# Autodesk Inventor assembly: NEMA 17 with T5 Pulley
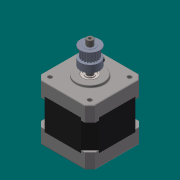
[picture p0: Inventor's stored thumbnail of the model, 180x180]
Saved by Autodesk Inventor 2016 (Build 200138000, 138)
## iProperties
Created: 2015-02-28
Part Number: NEMA 17 with T5 Pulley
Document SubType Name: Assembly
Designer: Sawaiz Syed
Title: NEMA 17 with T5 Pulley.STP
Description: STEP AP214
Creation Date: 2013-02-23
Sending System: SolidWorks 2012
Preprocessor: SwSTEP 2.0
Author: Sawaiz Syed
## Documents named in this file (8)
- C:\Users\Sawaiz\Documents\data\projects\cncBlackBox\nema17Stepper\nema17t5.iam
- C:\Users\Sawaiz\Documents\data\projects\cncBlackBox\nema17Stepper\stepperBase.ipt
- C:\Users\Sawaiz\Documents\data\projects\cncBlackBox\nema17Stepper\stepperBody.ipt
- C:\Users\Sawaiz\Documents\data\projects\cncBlackBox\nema17Stepper\stepperTop.ipt
- C:\Users\Sawaiz\Documents\data\projects\cncBlackBox\nema17Stepper\stepperScrews.ipt
- C:\Users\Sawaiz\Documents\data\projects\cncBlackBox\nema17Stepper\stepperShaft.ipt
- C:\Users\Sawaiz\Documents\data\projects\cncBlackBox\nema17Stepper\stepperBearing.ipt
- C:\Users\Sawaiz\Documents\data\projects\cncBlackBox\nema17Stepper\20tgt2Pulley.ipt
## Components (11 placed, 11 different names)
1. Base_1 — Mate:5, Mate:6, Mate:7, Flush:2, Flush:3, Mate:9, Mate:10, Mate:11, Mate:12, Mate:13
2. Cuerpo_2 — Mate:7, Flush:2, Flush:3, Flush:4, Flush:5, Mate:8
3. Tapa_3 — Mate:3, Flush:1, Flush:4, Flush:5, Mate:8
4. pan cross head_am_B18.6.7M - M3 x 0.5 x 5 Type I Cross Recessed PHMS --5N_4 — Mate:11, Flush:9, Flush:10, Mate:13
5. pan cross head_am_B18.6.7M - M3 x 0.5 x 5 Type I Cross Recessed PHMS --5N_5 — Mate:12, Flush:8, Flush:9
6. pan cross head_am_B18.6.7M - M3 x 0.5 x 5 Type I Cross Recessed PHMS --5N_6 — Mate:9, Flush:8
7. pan cross head_am_B18.6.7M - M3 x 0.5 x 5 Type I Cross Recessed PHMS --5N_7 — Mate:10, Flush:10
8. Eje_8 — Mate:4, Flush:6, Mate:14, Flush:11
9. instrument ball bearing_68_am_AFBMA 12.1.4.1 - 0050-11 - 10,SI,NC,10_68_9 — Mate:3, Flush:1, Mate:4
10. instrument ball bearing_68_am_AFBMA 12.1.4.1 - 0050-11 - 10,SI,NC,10_68_10 — Mate:5, Mate:6, Flush:6
11. T5 Pulley_12 — Mate:14, Flush:11
## Relationships (22: Mate 12, Flush 10)
- Mate:3: Tapa_3 ↔ instrument ball bearing_68_am_AFBMA 12.1.4.1 - 0050-11 - 10,SI,NC,10_68_9
- Flush:1: Tapa_3 ↔ instrument ball bearing_68_am_AFBMA 12.1.4.1 - 0050-11 - 10,SI,NC,10_68_9
- Mate:4: Eje_8 ↔ instrument ball bearing_68_am_AFBMA 12.1.4.1 - 0050-11 - 10,SI,NC,10_68_9
- Mate:5: Base_1 ↔ instrument ball bearing_68_am_AFBMA 12.1.4.1 - 0050-11 - 10,SI,NC,10_68_10
- Mate:6: Base_1 ↔ instrument ball bearing_68_am_AFBMA 12.1.4.1 - 0050-11 - 10,SI,NC,10_68_10
- Mate:7: Base_1 ↔ Cuerpo_2
- Flush:2: Base_1 ↔ Cuerpo_2
- Flush:3: Base_1 ↔ Cuerpo_2
- Flush:4: Cuerpo_2 ↔ Tapa_3
- Flush:5: Cuerpo_2 ↔ Tapa_3
- Mate:8: Cuerpo_2 ↔ Tapa_3
- Flush:6: Eje_8 ↔ instrument ball bearing_68_am_AFBMA 12.1.4.1 - 0050-11 - 10,SI,NC,10_68_10
- Mate:9: Base_1 ↔ pan cross head_am_B18.6.7M - M3 x 0.5 x 5 Type I Cross Recessed PHMS --5N_6
- Mate:10: Base_1 ↔ pan cross head_am_B18.6.7M - M3 x 0.5 x 5 Type I Cross Recessed PHMS --5N_7
- Mate:11: Base_1 ↔ pan cross head_am_B18.6.7M - M3 x 0.5 x 5 Type I Cross Recessed PHMS --5N_4
- Mate:12: Base_1 ↔ pan cross head_am_B18.6.7M - M3 x 0.5 x 5 Type I Cross Recessed PHMS --5N_5
- Flush:8: pan cross head_am_B18.6.7M - M3 x 0.5 x 5 Type I Cross Recessed PHMS --5N_5 ↔ pan cross head_am_B18.6.7M - M3 x 0.5 x 5 Type I Cross Recessed PHMS --5N_6
- Flush:9: pan cross head_am_B18.6.7M - M3 x 0.5 x 5 Type I Cross Recessed PHMS --5N_4 ↔ pan cross head_am_B18.6.7M - M3 x 0.5 x 5 Type I Cross Recessed PHMS --5N_5
- Flush:10: pan cross head_am_B18.6.7M - M3 x 0.5 x 5 Type I Cross Recessed PHMS --5N_4 ↔ pan cross head_am_B18.6.7M - M3 x 0.5 x 5 Type I Cross Recessed PHMS --5N_7
- Mate:13: Base_1 ↔ pan cross head_am_B18.6.7M - M3 x 0.5 x 5 Type I Cross Recessed PHMS --5N_4
- Mate:14: Eje_8 ↔ T5 Pulley_12
- Flush:11 (4.5 mm): Eje_8 ↔ T5 Pulley_12
